# Autodesk Inventor assembly: Robot Triciclo - Ensamble
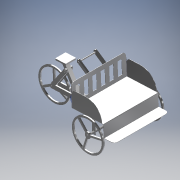
[picture p0: Inventor's stored thumbnail of the model, 180x180]
Saved by Autodesk Inventor 2019 (Build 230136000, 136)
## iProperties
Created: 2019-11-14
Part Number: Robot Triciclo - Ensamble
Document SubType Name: Weldment
Designer: eddysanoli
Weld Material: Welded Aluminum-6061
Author: eddysanoli
## Documents named in this file (13)
- C:\Users\Domenico\Documents\Inventor\Mecanismos2\Robot Triciclo - Ensamble.iam
- C:\Users\Domenico\Documents\Inventor\Mecanismos2\Asiento - Ensamble.iam
- C:\Users\Domenico\Documents\Inventor\Mecanismos2\Marco_triciclo.iam
- C:\Users\Domenico\Documents\Inventor\Mecanismos2\Rueda_triciclo.ipt
- C:\Users\Domenico\Documents\Inventor\Mecanismos2\Pedal.ipt
- C:\Users\Domenico\Documents\Inventor\Mecanismos2\Robot Triciclo - Ensamble\Design Accelerator\Eje1.iam
- C:\Users\Domenico\Documents\Inventor\Mecanismos2\Marco - Asiento Triciclo.ipt
- C:\Users\Domenico\Documents\Inventor\Mecanismos2\Robot Triciclo - Ensamble\Design Accelerator\Chain Drive1.iam
- C:\Users\Domenico\Documents\Inventor\Mecanismos2\Robot Triciclo - Ensamble\Design Accelerator\Eje Pedales - Ensamblaje.iam
- C:\Users\Domenico\Documents\Inventor\Mecanismos2\Robot Triciclo - Ensamble\Design Accelerator\Eje Pedales - Ensamblaje1.iam
- C:\Users\Domenico\Documents\Inventor\Mecanismos2\Robot Triciclo - Ensamble\Design Accelerator\Eje silla - Interno2.iam
- C:\Users\Domenico\Documents\Inventor\Mecanismos2\Robot Triciclo - Ensamble\Design Accelerator\Eje motor- Interno1.iam
- C:\Users\Domenico\Documents\Inventor\Mecanismos2\Robot Triciclo - Ensamble\Design Accelerator\Caja Reductora1.iam
## Components (14 placed, 12 different names)
1. Asiento - Ensamble:1 [sub-assembly] — Coincidencia:1, Coincidencia:2, Nivelación:1, Coincidencia:3, Coincidencia:4, Coincidencia:5, Coincidencia:6, Coincidencia:10
2. Marco_triciclo:2 [sub-assembly] — Coincidencia:1, Coincidencia:2, Nivelación:1, Coincidencia:7, Coincidencia:8, Coincidencia:9, Coincidencia:11, Nivelación:4, Nivelación:5, Mate:16, Mate:29, Mate:30, Angle:1, Mate:31, Mate:32, Angle:2, Mate:34, Mate:36, Mate:38, Flush:8
3. Rueda_triciclo:1 — Coincidencia:3, Coincidencia:5
4. Rueda_triciclo:2 — Coincidencia:4, Coincidencia:6
5. Pedal:1 — Nivelación:2, Coincidencia:7, Coincidencia:9, Flush:6
6. Pedal:2 — Nivelación:2, Coincidencia:8, Flush:7
7. Eje:1 [sub-assembly] — Coincidencia:10, Mate:35
8. Marco - Asiento Triciclo:1 — Coincidencia:11, Nivelación:4, Nivelación:5
9. Chain Drive:1 [sub-assembly] — Mate:17, Mate:37
10. Eje Pedales - Ensamblaje:1 [sub-assembly] — Mate:16, Flush:6, Flush:7, Mate:17, Mate:37
11. Eje Rueda Trasera - Ensamblaje:1 [sub-assembly] — Mate:38, Flush:8
12. Eje silla - Interno:1 [sub-assembly] — Mate:29, Mate:30, Angle:1
13. Eje motor - Interno:1 [sub-assembly] — Mate:31, Mate:32, Angle:2, Mate:33
14. Caja Reductora:1 [sub-assembly] — Mate:33, Mate:34, Mate:35, Mate:36
## Relationships (32: Mate 23, Flush 7, Angle 2)
- Coincidencia:1 [Mate]: Asiento - Ensamble:1 ↔ Marco_triciclo:2
- Coincidencia:2 [Mate] (59.8 mm): Asiento - Ensamble:1 ↔ Marco_triciclo:2
- Nivelación:1 [Flush] (183.5 mm): Asiento - Ensamble:1 ↔ Marco_triciclo:2
- Coincidencia:3 [Mate]: Asiento - Ensamble:1 ↔ Rueda_triciclo:1
- Coincidencia:4 [Mate]: Asiento - Ensamble:1 ↔ Rueda_triciclo:2
- Coincidencia:5 [Mate] (35 mm): Asiento - Ensamble:1 ↔ Rueda_triciclo:1
- Coincidencia:6 [Mate] (35 mm): Asiento - Ensamble:1 ↔ Rueda_triciclo:2
- Nivelación:2 [Flush]: Pedal:1 ↔ Pedal:2
- Coincidencia:7 [Mate]: Marco_triciclo:2 ↔ Pedal:1
- Coincidencia:8 [Mate]: Marco_triciclo:2 ↔ Pedal:2
- Coincidencia:9 [Mate]: Marco_triciclo:2 ↔ Pedal:1
- Coincidencia:10 [Mate]: Asiento - Ensamble:1 ↔ Eje:1
- Coincidencia:11 [Mate]: Marco_triciclo:2 ↔ Marco - Asiento Triciclo:1
- Nivelación:4 [Flush] (24 mm): Marco_triciclo:2 ↔ Marco - Asiento Triciclo:1
- Nivelación:5 [Flush] (-20 mm): Marco_triciclo:2 ↔ Marco - Asiento Triciclo:1
- Mate:16: Marco_triciclo:2 ↔ Eje Pedales - Ensamblaje:1
- Flush:6: Pedal:1 ↔ Eje Pedales - Ensamblaje:1
- Flush:7: Pedal:2 ↔ Eje Pedales - Ensamblaje:1
- Mate:17 (4.7 mm): Chain Drive:1 ↔ Eje Pedales - Ensamblaje:1
- Mate:29: Marco_triciclo:2 ↔ Eje silla - Interno:1
- Mate:30: Marco_triciclo:2 ↔ Eje silla - Interno:1
- Angle:1 (0 deg): Marco_triciclo:2 ↔ Eje silla - Interno:1
- Mate:31: Marco_triciclo:2 ↔ Eje motor - Interno:1
- Mate:32 (8.1245 mm): Marco_triciclo:2 ↔ Eje motor - Interno:1
- Angle:2 (0 deg): Marco_triciclo:2 ↔ Eje motor - Interno:1
- Mate:33: Eje motor - Interno:1 ↔ Caja Reductora:1
- Mate:34: Marco_triciclo:2 ↔ Caja Reductora:1
- Mate:35: Eje:1 ↔ Caja Reductora:1
- Mate:36: Marco_triciclo:2 ↔ Caja Reductora:1
- Mate:37: Chain Drive:1 ↔ Eje Pedales - Ensamblaje:1
- Mate:38: Marco_triciclo:2 ↔ Eje Rueda Trasera - Ensamblaje:1
- Flush:8: Marco_triciclo:2 ↔ Eje Rueda Trasera - Ensamblaje:1
